# Autodesk Inventor assembly: !tower
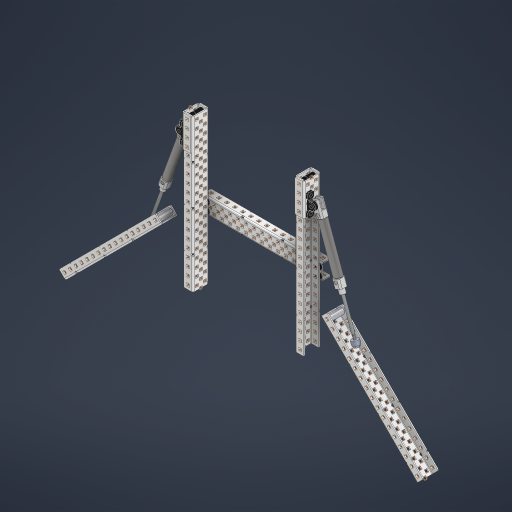
[picture p0: Inventor's stored thumbnail of the model, 512x512]
Saved by Autodesk Inventor 2024 (Build 280153000, 153)
## iProperties
Created: 2024-01-16
Part Number: !tower
Document SubType Name: Assembly
Designer: Averey Ku
Author: Averey Ku
## Documents named in this file (4)
- D:\vex_robotics\hardware\cad\zoomba_v0.3\tower\!tower.iam
- D:\vex_robotics\hardware\cad\zoomba_v0.3\tower\side.iam
- D:\vex_robotics\hardware\cad\zoomba_v0.3\tower\mirrored_parts\tower_MIR.iam
- D:\vex_robotics\hardware\cad\VEX-CAD-Inventor-1.41\Structure\C Channel\Aluminum 1x2x1\Alu C 1x2x1x15.ipt
## Components (3 placed, 3 different names)
1. side:1 [sub-assembly] — Insert:1, Mate:1
2. tower_MIR:1 [sub-assembly] — Insert:2
3. Alu C 1x2x1x15:1 — Insert:1, Mate:1, Insert:2
## Relationships (3: Insert 2, Mate 1)
- Insert:1: side:1 ↔ Alu C 1x2x1x15:1
- Mate:1: side:1 ↔ Alu C 1x2x1x15:1
- Insert:2: tower_MIR:1 ↔ Alu C 1x2x1x15:1
